# Autodesk Inventor assembly: cajas_V2
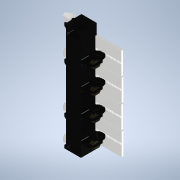
[picture p0: Inventor's stored thumbnail of the model, 180x180]
Saved by Autodesk Inventor 2022 (Build 260153000, 153)
## iProperties
Created: 2021-03-06
Part Number: cajas_V2
Document SubType Name: Assembly
Designer: juanp
Author: juanp
## Documents named in this file (7)
- C:\Users\juanp\OneDrive - Universidad de los andes\Uniandes\Robocol\EVA\V3 (Actual)\Cajas\cajas_V3.iam
- C:\Users\juanp\OneDrive - Universidad de los andes\Uniandes\Robocol\EVA\V3 (Actual)\Cajas\cajas_V3.ipt
- C:\Users\juanp\OneDrive - Universidad de los andes\Uniandes\Robocol\EVA\V3 (Actual)\Cajas\Engranaje V2.ipt
- C:\Users\juanp\OneDrive - Universidad de los andes\Uniandes\Robocol\EVA\V3 (Actual)\Cajas\Puerta Cremallera V3.ipt
- C:\Users\juanp\OneDrive - Universidad de los andes\Uniandes\Robocol\EVA\Recursos\Servo MG90S\MG90S.iam
- C:\Users\juanp\OneDrive - Universidad de los andes\Uniandes\Robocol\EVA\V3 (Actual)\Cajas\Soporte motor.ipt
- C:\Users\juanp\OneDrive - Universidad de los andes\Uniandes\Robocol\EVA\Recursos\Servo MG90S\attachment.ipt
## Components (21 placed, 6 different names)
1. cajas_V3:1 — Mate:6, Mate:7, Mate:8, Mate:9, Mate:10, Mate:13, Angle:1, Mate:30, Mate:31, Mate:32, Mate:33, Flush:1, Mate:34, Mate:35, Mate:36, Mate:37, Mate:38, Mate:39, Mate:40, Mate:41, Flush:2, Mate:42, Flush:3, Mate:43, Mate:44, Mate:45, Flush:7
2. Engranaje V2:1 — Rotation/Translation:1, Mate:14, Mate:15, Angle:2
3. Puerta Cremallera V3:1 — Mate:6, Mate:7, Rotation/Translation:1
4. MG90S:1 [sub-assembly] — Mate:8, Mate:9, Mate:10, Mate:16, Mate:17
5. Soporte motor:1 — Mate:13, Angle:1, Flush:3, Flush:4
6. attachment:1 — Mate:14, Mate:15, Angle:2, Mate:16, Mate:17
7. Engranaje V2:2
8. Puerta Cremallera V3:2 — Mate:33, Flush:1
9. MG90S:2 [sub-assembly] — Mate:30, Mate:31, Mate:32
10. attachment:2
11. Engranaje V2:3
12. Puerta Cremallera V3:3 — Mate:40, Mate:42
13. MG90S:3 [sub-assembly] — Mate:34, Mate:35, Mate:36
14. attachment:3
15. Engranaje V2:4
16. Puerta Cremallera V3:4 — Mate:41, Flush:2
17. MG90S:4 [sub-assembly] — Mate:37, Mate:38, Mate:39
18. attachment:4
19. Soporte motor:2 — Flush:5, Flush:6, Mate:44
20. Soporte motor:3 — Flush:4, Flush:5, Mate:45, Flush:7
21. Soporte motor:4 — Flush:6, Mate:43
## Relationships (54: Mate 38, Flush 7, Angle 5, RelateRotateTranslate 4)
- Mate:6: cajas_V3:1 ↔ Puerta Cremallera V3:1
- Mate:7: cajas_V3:1 ↔ Puerta Cremallera V3:1
- Mate:8: cajas_V3:1 ↔ MG90S:1
- Mate:9: cajas_V3:1 ↔ MG90S:1
- Mate:10: cajas_V3:1 ↔ MG90S:1
- Rotation/Translation:1 [RelateRotateTranslate] (125.664 mm): Engranaje V2:1 ↔ Puerta Cremallera V3:1
- Mate:13: cajas_V3:1 ↔ Soporte motor:1
- Angle:1 (180 deg): cajas_V3:1 ↔ Soporte motor:1
- Mate:14: Engranaje V2:1 ↔ attachment:1
- Mate:15: Engranaje V2:1 ↔ attachment:1
- Angle:2 (0 deg): Engranaje V2:1 ↔ attachment:1
- Mate:16: MG90S:1 ↔ attachment:1
- Mate:17: MG90S:1 ↔ attachment:1
- [RelateRotateTranslate] (125.664 mm): Engranaje V2:2 ↔ Puerta Cremallera V3:2
- [Mate]: Engranaje V2:2 ↔ attachment:2
- [Mate]: Engranaje V2:2 ↔ attachment:2
- [Angle] (0 deg): Engranaje V2:2 ↔ attachment:2
- [Mate]: MG90S:2 ↔ attachment:2
- [Mate]: MG90S:2 ↔ attachment:2
- [RelateRotateTranslate] (125.664 mm): Engranaje V2:3 ↔ Puerta Cremallera V3:3
- [Mate]: Engranaje V2:3 ↔ attachment:3
- [Mate]: Engranaje V2:3 ↔ attachment:3
- [Angle] (0 deg): Engranaje V2:3 ↔ attachment:3
- [Mate]: MG90S:3 ↔ attachment:3
- [Mate]: MG90S:3 ↔ attachment:3
- [RelateRotateTranslate] (125.664 mm): Engranaje V2:4 ↔ Puerta Cremallera V3:4
- [Mate]: Engranaje V2:4 ↔ attachment:4
- [Mate]: Engranaje V2:4 ↔ attachment:4
- [Angle] (0 deg): Engranaje V2:4 ↔ attachment:4
- [Mate]: MG90S:4 ↔ attachment:4
- [Mate]: MG90S:4 ↔ attachment:4
- Mate:30: cajas_V3:1 ↔ MG90S:2
- Mate:31: cajas_V3:1 ↔ MG90S:2
- Mate:32: cajas_V3:1 ↔ MG90S:2
- Mate:33: cajas_V3:1 ↔ Puerta Cremallera V3:2
- Flush:1: cajas_V3:1 ↔ Puerta Cremallera V3:2
- Mate:34: cajas_V3:1 ↔ MG90S:3
- Mate:35: cajas_V3:1 ↔ MG90S:3
- Mate:36: cajas_V3:1 ↔ MG90S:3
- Mate:37: cajas_V3:1 ↔ MG90S:4
- Mate:38: cajas_V3:1 ↔ MG90S:4
- Mate:39: cajas_V3:1 ↔ MG90S:4
- Mate:40: cajas_V3:1 ↔ Puerta Cremallera V3:3
- Mate:41: cajas_V3:1 ↔ Puerta Cremallera V3:4
- Flush:2: cajas_V3:1 ↔ Puerta Cremallera V3:4
- Mate:42: cajas_V3:1 ↔ Puerta Cremallera V3:3
- Flush:3: cajas_V3:1 ↔ Soporte motor:1
- Flush:4: Soporte motor:1 ↔ Soporte motor:3
- Flush:5: Soporte motor:2 ↔ Soporte motor:3
- Flush:6: Soporte motor:2 ↔ Soporte motor:4
- Mate:43: cajas_V3:1 ↔ Soporte motor:4
- Mate:44: cajas_V3:1 ↔ Soporte motor:2
- Mate:45: cajas_V3:1 ↔ Soporte motor:3
- Flush:7: cajas_V3:1 ↔ Soporte motor:3
## Named parameters: d36_d19 = 125.664 mm, d37_d31 = 0 mm, d38_d32 = 0 mm, d39_d33 = 0 deg, d40_d34 = 0 mm, d41_d35 = 0 mm, d42_d19 = 125.664 mm, d43_d31 = 0 mm, d44_d32 = 0 mm, d45_d33 = 0 deg, d46_d34 = 0 mm, d47_d35 = 0 mm, d48_d19 = 125.664 mm, d49_d31 = 0 mm, d50_d32 = 0 mm, d51_d33 = 0 deg, d52_d34 = 0 mm, d53_d35 = 0 mm
